# Autodesk Inventor assembly: SensorAssembly
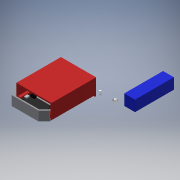
[picture p0: Inventor's stored thumbnail of the model, 180x180]
Saved by Autodesk Inventor 2018 (Build 220112000, 112)
## iProperties
Created: 2019-10-14
Part Number: SensorAssembly
Document SubType Name: Assembly
Designer: jklei
Author: jklei
## Documents named in this file (6)
- C:\Users\jklei\Desktop\Wildfire-Detector\CAD\SensorAssembly.iam
- C:\Users\jklei\Desktop\Wildfire-Detector\CAD\2829 Adafruit Feather Bluefruit 32u4.ipt
- C:\Users\jklei\Desktop\Wildfire-Detector\CAD\sensor.ipt
- C:\Users\jklei\Desktop\Wildfire-Detector\CAD\bottom-housing.ipt
- C:\Users\jklei\Desktop\Wildfire-Detector\CAD\top-slider.ipt
- C:\Users\jklei\Desktop\Wildfire-Detector\CAD\Battery.ipt
## Components (6 placed, 5 different names)
1. 2829 Adafruit Feather Bluefruit 32u4:1 — Mate:4, Mate:5, Flush:2
2. sensor:1
3. sensor:2
4. bottom-housing:1 — Mate:4, Mate:5, Flush:1, Flush:2
5. top-slider:1 — Flush:1
6. Battery:1
## Relationships (4: Mate 2, Flush 2)
- Mate:4 (6.35 mm): 2829 Adafruit Feather Bluefruit 32u4:1 ↔ bottom-housing:1
- Mate:5 (9.525 mm): 2829 Adafruit Feather Bluefruit 32u4:1 ↔ bottom-housing:1
- Flush:1: bottom-housing:1 ↔ top-slider:1
- Flush:2 (12.7 mm): 2829 Adafruit Feather Bluefruit 32u4:1 ↔ bottom-housing:1
